# Autodesk Inventor assembly: Ensamblaje1
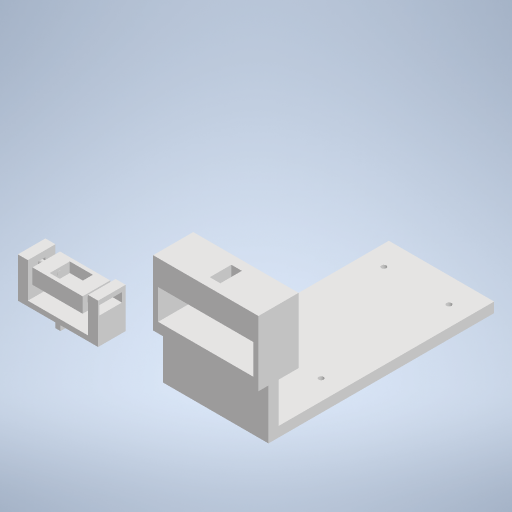
[picture p0: Inventor's stored thumbnail of the model, 512x512]
Saved by Autodesk Inventor 2023 (Build 270158000, 158)
## iProperties
Created: 2022-07-04
Part Number: Ensamblaje1
Document SubType Name: Assembly
Designer: inigo
Author: inigo
## Documents named in this file (5)
- D:\projects\FoBo\model\Ensamblaje1.iam
- D:\projects\FoBo\model\base.ipt
- D:\projects\FoBo\model\camera_support.ipt
- D:\projects\FoBo\model\camera_support_2.ipt
- D:\projects\FoBo\model\camera_support_union.ipt
## Components (4 placed, 4 different names)
1. base:1
2. camera_support:1
3. camera_support_2:1 — Coincidencia:1
4. camera_support_union:1 — Coincidencia:1
## Relationships (1: Mate 1)
- Coincidencia:1 [Mate]: camera_support_2:1 ↔ camera_support_union:1
